# Autodesk Inventor assembly: Assembly2
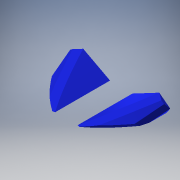
[picture p0: Inventor's stored thumbnail of the model, 180x180]
Saved by Autodesk Inventor 2016 (Build 200138000, 138)
## iProperties
Created: 2015-06-02
Part Number: Assembly2
Document SubType Name: Assembly
Designer: Spooner
Author: Spooner
## Documents named in this file (3)
- C:\Users\Spooner\Documents\Inventor\RoboCat Gen 2\Assembly2.iam
- C:\Users\Spooner\Documents\Inventor\RoboCat Gen 2\Cat.ipt
- C:\Users\Spooner\Documents\Inventor\RoboCat Gen 2\Eyes.ipt
## Components (2 placed, 2 different names)
1. Cat:1 — Mate:1, Angle:1, Mate:2, Mate:3, Mate:4, Mate:5, Mate:6
2. Eyes:1 — Mate:4, Mate:5, Mate:6
## Relationships (7: Mate 6, Angle 1)
- Mate:1: Cat:1
- Angle:1 (0 deg): Cat:1
- Mate:2 (-6.35 mm): Cat:1
- Mate:3: Cat:1
- Mate:4: Cat:1 ↔ Eyes:1
- Mate:5: Cat:1 ↔ Eyes:1
- Mate:6: Cat:1 ↔ Eyes:1
